# Autodesk Inventor assembly: Box_Assembly_1
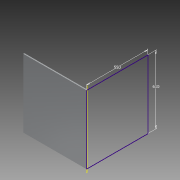
[picture p0: Inventor's stored thumbnail of the model, 180x180]
Saved by Autodesk Inventor 2015 SP2 (Build 190223200, 223)
## iProperties
Created: 2016-11-10
Part Number: Box_Assembly_1
Document SubType Name: Assembly
Designer: Yann Cesbron
Mass: 17001 g
Surface Area: 35169 cm^2
Volume: 17001 cm^3
Density: 1 g/cm^3
Author: Yann Cesbron
## Documents named in this file (3)
- C:\Yann\Docs\Materials\DIY stuffs\PALM_scope_incubation_box\Box_Assembly_1.iam
- C:\Yann\Docs\Materials\DIY stuffs\PALM_scope_incubation_box\Box_front.ipt
- C:\Yann\Docs\Materials\DIY stuffs\Right side.ipt
## Components (2 placed, 2 different names)
1. Box_front:1 — Flush:1, Flush:3
2. Right side:1 — Flush:1, Flush:3
## Relationships (2: Flush 2)
- Flush:1: Box_front:1 ↔ Right side:1
- Flush:3: Box_front:1 ↔ Right side:1
